# Autodesk Inventor assembly: y_carriage_assembly
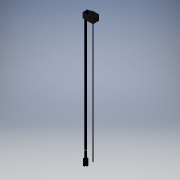
[picture p0: Inventor's stored thumbnail of the model, 180x180]
Saved by Autodesk Inventor 2018 (Build 220112000, 112)
## iProperties
Created: 2017-11-16
Part Number: y_carriage_assembly
Document SubType Name: Assembly
Designer: g
Author: g
## Documents named in this file (8)
- C:\Users\g\Desktop\AUG_inventor\y_carriage_assembly.iam
- C:\Users\g\Desktop\AUG_inventor\M3 X 10mm Screw.ipt
- C:\Users\g\Desktop\AUG_inventor\NEMA17 w connector metric.ipt
- C:\Users\g\Desktop\AUG_inventor\8M 900mm threaded rod.ipt
- C:\Users\g\Desktop\AUG_inventor\makerbeam1000mm.ipt
- C:\Users\g\Desktop\AUG_inventor\5mm to 8mm holder.ipt
- C:\Users\g\Desktop\AUG_inventor\makerbeam40mm.ipt
- C:\Users\g\Desktop\AUG_inventor\nema 17 holder.ipt
## Components (17 placed, 7 different names)
1. 8M 900mm threaded rod:1 — Rigid:8, Mate:309, Mate:310, Mate:311
2. makerbeam1000mm:1 — Flush:172, Mate:288, Mate:289, Flush:173, Flush:174, Flush:175, Flush:176, Mate:300, Flush:179, Flush:180, Flush:181, Flush:182, Mate:301, Flush:183, Mate:302, Flush:184, Mate:303, Mate:304, Flush:185, Flush:186
3. NEMA17 w connector metric:4 — Flush:172, Mate:307, Mate:308, Mate:309, Mate:310, Mate:311
4. 5mm to 8mm holder:1 — Rigid:8
5. makerbeam40mm:1 — Mate:288, Flush:174, Flush:175, Flush:177, Flush:178
6. makerbeam40mm:2 — Mate:289, Flush:173, Flush:176, Mate:293
7. nema 17 holder:1 — Flush:177, Flush:178, Mate:293, Cylindrical:124, Cylindrical:125, Cylindrical:126, Mate:294, Mate:295, Mate:296, Cylindrical:127, Cylindrical:128, Cylindrical:129, Mate:297, Mate:298, Mate:299, Mate:307, Mate:308
8. M3 X 10mm Screw:53 — Cylindrical:124, Mate:294
9. M3 X 10mm Screw:54 — Cylindrical:127, Mate:299
10. M3 X 10mm Screw:55 — Cylindrical:128, Mate:298
11. M3 X 10mm Screw:56 — Cylindrical:129, Mate:297
12. M3 X 10mm Screw:57 — Cylindrical:126, Mate:296
13. M3 X 10mm Screw:58 — Cylindrical:125, Mate:295
14. makerbeam40mm:3 — Flush:183, Mate:302, Flush:184, Mate:303
15. makerbeam40mm:4 — Mate:304, Flush:185, Flush:186
16. makerbeam40mm:5 — Mate:300, Flush:179, Flush:180
17. makerbeam40mm:6 — Flush:181, Flush:182, Mate:301
## Relationships (41: Mate 19, Flush 15, CylindricalJoint 6, WeldJoint 1)
- Rigid:8 [WeldJoint] (-12 mm): 8M 900mm threaded rod:1 ↔ 5mm to 8mm holder:1
- Flush:172: makerbeam1000mm:1 ↔ NEMA17 w connector metric:4
- Mate:288: makerbeam1000mm:1 ↔ makerbeam40mm:1
- Mate:289: makerbeam1000mm:1 ↔ makerbeam40mm:2
- Flush:173: makerbeam1000mm:1 ↔ makerbeam40mm:2
- Flush:174: makerbeam1000mm:1 ↔ makerbeam40mm:1
- Flush:175: makerbeam1000mm:1 ↔ makerbeam40mm:1
- Flush:176: makerbeam1000mm:1 ↔ makerbeam40mm:2
- Flush:177: makerbeam40mm:1 ↔ nema 17 holder:1
- Flush:178: makerbeam40mm:1 ↔ nema 17 holder:1
- Mate:293: makerbeam40mm:2 ↔ nema 17 holder:1
- Cylindrical:124: nema 17 holder:1 ↔ M3 X 10mm Screw:53
- Cylindrical:125: nema 17 holder:1 ↔ M3 X 10mm Screw:58
- Cylindrical:126: nema 17 holder:1 ↔ M3 X 10mm Screw:57
- Mate:294: nema 17 holder:1 ↔ M3 X 10mm Screw:53
- Mate:295: nema 17 holder:1 ↔ M3 X 10mm Screw:58
- Mate:296: nema 17 holder:1 ↔ M3 X 10mm Screw:57
- Cylindrical:127: nema 17 holder:1 ↔ M3 X 10mm Screw:54
- Cylindrical:128: nema 17 holder:1 ↔ M3 X 10mm Screw:55
- Cylindrical:129: nema 17 holder:1 ↔ M3 X 10mm Screw:56
- Mate:297: nema 17 holder:1 ↔ M3 X 10mm Screw:56
- Mate:298: nema 17 holder:1 ↔ M3 X 10mm Screw:55
- Mate:299: nema 17 holder:1 ↔ M3 X 10mm Screw:54
- Mate:300: makerbeam1000mm:1 ↔ makerbeam40mm:5
- Flush:179: makerbeam1000mm:1 ↔ makerbeam40mm:5
- Flush:180: makerbeam1000mm:1 ↔ makerbeam40mm:5
- Flush:181: makerbeam1000mm:1 ↔ makerbeam40mm:6
- Flush:182: makerbeam1000mm:1 ↔ makerbeam40mm:6
- Mate:301: makerbeam1000mm:1 ↔ makerbeam40mm:6
- Flush:183: makerbeam1000mm:1 ↔ makerbeam40mm:3
- Mate:302: makerbeam1000mm:1 ↔ makerbeam40mm:3
- Flush:184: makerbeam1000mm:1 ↔ makerbeam40mm:3
- Mate:303: makerbeam1000mm:1 ↔ makerbeam40mm:3
- Mate:304: makerbeam1000mm:1 ↔ makerbeam40mm:4
- Flush:185: makerbeam1000mm:1 ↔ makerbeam40mm:4
- Flush:186: makerbeam1000mm:1 ↔ makerbeam40mm:4
- Mate:307: NEMA17 w connector metric:4 ↔ nema 17 holder:1
- Mate:308: NEMA17 w connector metric:4 ↔ nema 17 holder:1
- Mate:309: 8M 900mm threaded rod:1 ↔ NEMA17 w connector metric:4
- Mate:310: 8M 900mm threaded rod:1 ↔ NEMA17 w connector metric:4
- Mate:311: 8M 900mm threaded rod:1 ↔ NEMA17 w connector metric:4
